# Autodesk Inventor assembly: リンク_ふともも_前_1
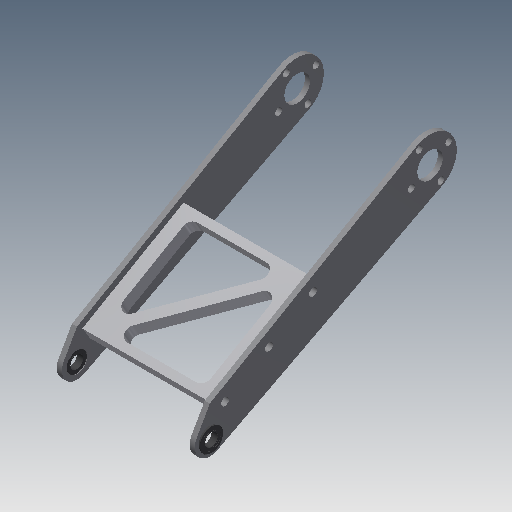
[picture p0: Inventor's stored thumbnail of the model, 512x512]
Saved by Autodesk Inventor 2017.3 (Build 213256000, 256)
## iProperties
Created: 2016-04-27
Part Number: リンク_ふともも_前_1
Document SubType Name: Assembly
Designer: hiroaki
Mass: 43.9245 g
Surface Area: 135.344 cm^2
Volume: 11.595 cm^3
Density: 3.78822 g/cm^3
Author: hiroaki
## Documents named in this file (4)
- C:\Users\haya\Desktop\GankenKun0_5\下半身\リンク\ふともも\リンク_ふともも_前_1.iam
- C:\Users\haya\Desktop\GankenKun0_5\下半身\リンク\ふともも\リンク_ふともも_メインフレーム_1_1.ipt
- C:\Users\haya\Desktop\GankenKun0_5\既製品\NSK_RB_MF85ZZ\MF85ZZ.iam
- C:\Users\haya\Desktop\GankenKun0_5\下半身\リンク\ふともも\リンク_ふともも_サブフレーム_1_1(予備案).ipt
## Components (5 placed, 3 different names)
1. リンク_ふともも_メインフレーム_1_1:1 — 挿入:13, 挿入:18, 挿入:19, 挿入:20
2. リンク_ふともも_メインフレーム_1_1:2 — 挿入:14, 挿入:15, 挿入:16, 挿入:17
3. MF85ZZ:1 [sub-assembly] — 挿入:13
4. MF85ZZ:2 [sub-assembly] — 挿入:14
5. リンク_ふともも_サブフレーム_1_1(予備案):1 — 挿入:15, 挿入:16, 挿入:17, 挿入:18, 挿入:19, 挿入:20
## Relationships (8: Insert 8)
- 挿入:13 [Insert]: リンク_ふともも_メインフレーム_1_1:1 ↔ MF85ZZ:1
- 挿入:14 [Insert]: リンク_ふともも_メインフレーム_1_1:2 ↔ MF85ZZ:2
- 挿入:15 [Insert]: リンク_ふともも_メインフレーム_1_1:2 ↔ リンク_ふともも_サブフレーム_1_1(予備案):1
- 挿入:16 [Insert]: リンク_ふともも_メインフレーム_1_1:2 ↔ リンク_ふともも_サブフレーム_1_1(予備案):1
- 挿入:17 [Insert]: リンク_ふともも_メインフレーム_1_1:2 ↔ リンク_ふともも_サブフレーム_1_1(予備案):1
- 挿入:18 [Insert]: リンク_ふともも_メインフレーム_1_1:1 ↔ リンク_ふともも_サブフレーム_1_1(予備案):1
- 挿入:19 [Insert]: リンク_ふともも_メインフレーム_1_1:1 ↔ リンク_ふともも_サブフレーム_1_1(予備案):1
- 挿入:20 [Insert]: リンク_ふともも_メインフレーム_1_1:1 ↔ リンク_ふともも_サブフレーム_1_1(予備案):1
## Named parameters: sa_0 = -1.8667e-08, sa_1 = 24986.6, sa_2 = 818.566
note: some values were not read from the file. Shown as the stored number, unit unknown: "sa_0", "sa_1", "sa_2".
